# Autodesk Inventor assembly: R-W v6
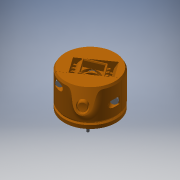
[picture p0: Inventor's stored thumbnail of the model, 180x180]
Saved by Autodesk Inventor 2018.2 (Build 222227000, 227)
## iProperties
Created: 2017-09-22
Part Number: R-W v6
Material: 一般
Document SubType Name: Assembly
Designer: sktom
Author: sktom
## Documents named in this file (14)
- D:\CloudStrage\OneDrive\CADMech\HbSizeMMech\UnitWrist\Unit_MR-W.iam
- D:\CloudStrage\OneDrive\CADMech\HbSizeMMech\UnitWrist\MR-W-02.ipt
- D:\CloudStrage\OneDrive\CADMech\HbSizeMMech\UnitWrist\MR-W-01.ipt
- D:\CloudStrage\OneDrive\CADMech\HbSizeMMech\UnitWrist\MR-W-04.ipt
- D:\CloudStrage\OneDrive\CADMech\HbSizeMMech\UnitWrist\MR-W-05.ipt
- D:\CloudStrage\OneDrive\CADMech\HbSizeMMech\UnitWrist\MR-W-06.ipt
- D:\CloudStrage\OneDrive\CADMech\HbSizeMMech\UnitWrist\MR-W-07.ipt
- D:\CloudStrage\OneDrive\CADMech\HbSizeMMech\UnitWrist\MR-W-08.ipt
- D:\CloudStrage\OneDrive\CADMech\HbSizeMMech\UnitWrist\MR-W-03.ipt
- D:\CloudStrage\OneDrive\CADMech\HbSizeMMech\UnitWrist\Parts_CoilSpring_CS 0.29-5.5-8.ipt
- D:\CloudStrage\OneDrive\CADMech\HbSizeMMech\UnitWrist\Parts_FlatScrew_M2_L6.ipt
- D:\CloudStrage\OneDrive\CADMech\HbSizeMMech\UnitWrist\Parts_Screw_M3_L6.ipt
- D:\CloudStrage\OneDrive\CADMech\HbSizeMMech\UnitWrist\Parts_Screw_M2_L8.ipt
- D:\CloudStrage\OneDrive\CADMech\HbSizeMMech\UnitWrist\Parts_SBM-SUJ-5.5.ipt
## Components (21 placed, 13 different names)
1. R-W-01 v2:1 — 挿入:12, メイト:1, 挿入:13
2. R-W-02 v2:1 — 挿入:8, 円柱状:1, 円柱状:2, フラッシュ:1, 挿入:9, 挿入:10, 挿入:11, 挿入:12, メイト:1, 挿入:14, メイト:2, 挿入:15, 挿入:16
3. R-W-03 v1:1 — 円柱状:1, 円柱状:2, フラッシュ:1
4. R-W-04 v2:1 — 挿入:1, 挿入:2, 挿入:5, 挿入:6, 挿入:7, 挿入:8
5. R-W-05 v2:1 — 挿入:1, 挿入:2, 挿入:3, 挿入:4
6. R-W-06 v2:1 — 挿入:14, 円柱状:3
7. R-W-07 v2:1 — 円柱状:3, メイト:2
8. R-W-08 v2:1 — 挿入:15, 挿入:16, 挿入:17, 挿入:18
9. Parts_SBM-SUJ-5.5:1
10. Parts_SBM-SUJ-5.5:2
11. Parts_CoilSpring_CS 0.29-5.5-8:1 — 挿入:10
12. Parts_CoilSpring_CS 0.29-5.5-8:2 — 挿入:9
13. Parts_CoilSpring_CS 0.29-5.5-8:3 — 挿入:11
14. Parts_Screw_M3_L6:1 — 挿入:18
15. Parts_Screw_M3_L6:2 — 挿入:17
16. Parts_FlatScrew_M2_L6:1 — 挿入:4
17. Parts_FlatScrew_M2_L6:2 — 挿入:3
18. Parts_Screw_M2_L8:1 — 挿入:6
19. Parts_Screw_M2_L8:2 — 挿入:7
20. Parts_Screw_M2_L8:3 — 挿入:5
21. Parts_CoilSpring_CS 0.29-5.5-8:4 — 挿入:13
## Relationships (24: Insert 18, CylindricalJoint 3, Mate 2, Flush 1)
- 挿入:1 [Insert]: R-W-04 v2:1 ↔ R-W-05 v2:1
- 挿入:2 [Insert]: R-W-04 v2:1 ↔ R-W-05 v2:1
- 挿入:3 [Insert]: R-W-05 v2:1 ↔ Parts_FlatScrew_M2_L6:2
- 挿入:4 [Insert]: R-W-05 v2:1 ↔ Parts_FlatScrew_M2_L6:1
- 挿入:5 [Insert]: R-W-04 v2:1 ↔ Parts_Screw_M2_L8:3
- 挿入:6 [Insert]: R-W-04 v2:1 ↔ Parts_Screw_M2_L8:1
- 挿入:7 [Insert]: R-W-04 v2:1 ↔ Parts_Screw_M2_L8:2
- 挿入:8 [Insert]: R-W-02 v2:1 ↔ R-W-04 v2:1
- 円柱状:1 [CylindricalJoint]: R-W-02 v2:1 ↔ R-W-03 v1:1
- 円柱状:2 [CylindricalJoint]: R-W-02 v2:1 ↔ R-W-03 v1:1
- フラッシュ:1 [Flush]: R-W-02 v2:1 ↔ R-W-03 v1:1
- 挿入:9 [Insert]: R-W-02 v2:1 ↔ Parts_CoilSpring_CS 0.29-5.5-8:2
- 挿入:10 [Insert]: R-W-02 v2:1 ↔ Parts_CoilSpring_CS 0.29-5.5-8:1
- 挿入:11 [Insert]: R-W-02 v2:1 ↔ Parts_CoilSpring_CS 0.29-5.5-8:3
- 挿入:12 [Insert]: R-W-01 v2:1 ↔ R-W-02 v2:1
- メイト:1 [Mate] (0.265 mm): R-W-01 v2:1 ↔ R-W-02 v2:1
- 挿入:13 [Insert]: R-W-01 v2:1 ↔ Parts_CoilSpring_CS 0.29-5.5-8:4
- 挿入:14 [Insert]: R-W-02 v2:1 ↔ R-W-06 v2:1
- 円柱状:3 [CylindricalJoint]: R-W-06 v2:1 ↔ R-W-07 v2:1
- メイト:2 [Mate]: R-W-02 v2:1 ↔ R-W-07 v2:1
- 挿入:15 [Insert]: R-W-02 v2:1 ↔ R-W-08 v2:1
- 挿入:16 [Insert]: R-W-02 v2:1 ↔ R-W-08 v2:1
- 挿入:17 [Insert]: R-W-08 v2:1 ↔ Parts_Screw_M3_L6:2
- 挿入:18 [Insert]: R-W-08 v2:1 ↔ Parts_Screw_M3_L6:1
